# Autodesk Inventor assembly: Egg Capsule Complete
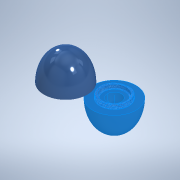
[picture p0: Inventor's stored thumbnail of the model, 180x180]
Saved by Autodesk Inventor 2022 (Build 260153000, 153)
## iProperties
Created: 2022-02-15
Part Number: Egg Capsule Complete
Document SubType Name: Assembly
Designer: Nathan Griffith
Author: Nathan Griffith
## Documents named in this file (3)
- C:\Users\Nathan Griffith\Documents\Inventor\Physics Egg Drop\Egg Capsule Complete.iam
- C:\Users\Nathan Griffith\Documents\Inventor\Physics Egg Drop\Egg Capsule ver 2 part 2.iam
- C:\Users\Nathan Griffith\Documents\Inventor\Physics Egg Drop\Egg Capsule ver 2.iam
## Components (2 placed, 2 different names)
1. Egg Capsule ver 2 part 2:1 [sub-assembly] — Insert:1
2. Egg Capsule ver 2:1 [sub-assembly] — Insert:1
## Relationships (1: Insert 1)
- Insert:1: Egg Capsule ver 2 part 2:1 ↔ Egg Capsule ver 2:1
